# Autodesk Inventor assembly: Assembly with Weights
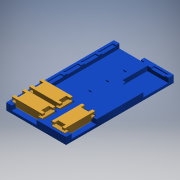
[picture p0: Inventor's stored thumbnail of the model, 180x180]
Saved by Autodesk Inventor 2019.4 (Build 234330000, 330)
## iProperties
Created: 2021-03-04
Part Number: Assembly with Weights
Document SubType Name: Assembly
Designer: caleb
Author: caleb
## Documents named in this file (3)
- C:\Users\cfang\Desktop\nebraska-silicon-lab\Hardware\ETL\Module Assembly\Glue Stamp Staging Plate\Assembly with Weights.iam
- C:\Users\cfang\Desktop\nebraska-silicon-lab\Hardware\ETL\Module Assembly\Weight\Weight Assembly.iam
- C:\Users\cfang\Desktop\nebraska-silicon-lab\Hardware\ETL\Module Assembly\Glue Stamp Staging Plate\Glue Stamp Staging Plate.ipt
## Components (4 placed, 2 different names)
1. Weight Assembly:1 [sub-assembly] — Mate:1, Mate:2, Mate:3
2. Glue Stamp Staging Plate:1 — Mate:1, Mate:2, Mate:3, Mate:4, Mate:5, Mate:6, Mate:7, Mate:8, Mate:9
3. Weight Assembly:2 [sub-assembly] — Mate:4, Mate:5, Mate:6
4. Weight Assembly:3 [sub-assembly] — Mate:7, Mate:8, Mate:9
## Relationships (9: Mate 9)
- Mate:1: Weight Assembly:1 ↔ Glue Stamp Staging Plate:1
- Mate:2: Weight Assembly:1 ↔ Glue Stamp Staging Plate:1
- Mate:3: Weight Assembly:1 ↔ Glue Stamp Staging Plate:1
- Mate:4: Glue Stamp Staging Plate:1 ↔ Weight Assembly:2
- Mate:5: Glue Stamp Staging Plate:1 ↔ Weight Assembly:2
- Mate:6: Glue Stamp Staging Plate:1 ↔ Weight Assembly:2
- Mate:7: Glue Stamp Staging Plate:1 ↔ Weight Assembly:3
- Mate:8: Glue Stamp Staging Plate:1 ↔ Weight Assembly:3
- Mate:9: Glue Stamp Staging Plate:1 ↔ Weight Assembly:3
